# Autodesk Inventor assembly: Module Cradle V1
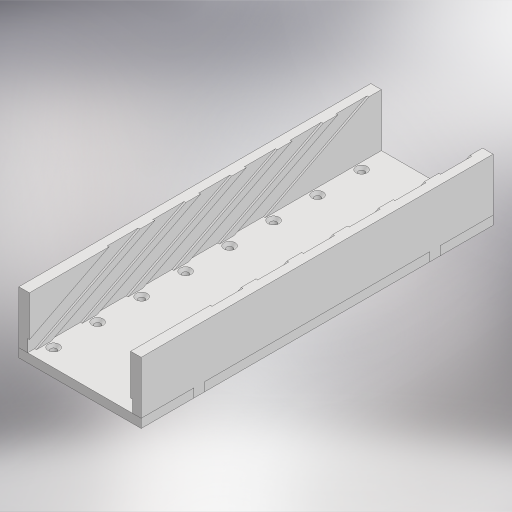
[picture p0: Inventor's stored thumbnail of the model, 512x512]
Saved by Autodesk Inventor 2024 (Build 280153000, 153)
## iProperties
Created: 2024-03-20
Part Number: Module Cradle V1
Document SubType Name: Assembly
Designer: cfang
Author: cfang
## Documents named in this file (4)
- C:\Users\cfang\Desktop\nebraska-silicon-lab\Hardware\ETL\Irradiation Fixture\Module Cradle V1.iam
- C:\Users\cfang\Desktop\nebraska-silicon-lab\Hardware\ETL\Irradiation Fixture\Module Cradle Left V1.ipt
- C:\Users\cfang\Desktop\nebraska-silicon-lab\Hardware\ETL\Irradiation Fixture\Module Cradle Base V1.ipt
- C:\Users\cfang\Desktop\nebraska-silicon-lab\Hardware\ETL\Irradiation Fixture\Module Cradle Right V1.ipt
## Components (3 placed, 3 different names)
1. Module Cradle Left V1:2 — Mate:1, Flush:1, Flush:2
2. Module Cradle Base V1:1 — Mate:1, Flush:1, Flush:2, Mate:2, Flush:3, Flush:4
3. Module Cradle Right V1:1 — Mate:2, Flush:3, Flush:4
## Relationships (6: Flush 4, Mate 2)
- Mate:1: Module Cradle Left V1:2 ↔ Module Cradle Base V1:1
- Flush:1: Module Cradle Left V1:2 ↔ Module Cradle Base V1:1
- Flush:2: Module Cradle Left V1:2 ↔ Module Cradle Base V1:1
- Mate:2: Module Cradle Base V1:1 ↔ Module Cradle Right V1:1
- Flush:3: Module Cradle Base V1:1 ↔ Module Cradle Right V1:1
- Flush:4: Module Cradle Base V1:1 ↔ Module Cradle Right V1:1
